# Autodesk Inventor assembly: X-axis assy
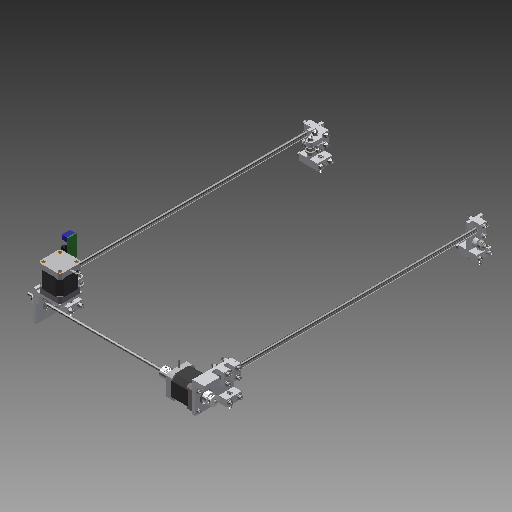
[picture p0: Inventor's stored thumbnail of the model, 512x512]
Saved by Autodesk Inventor 2018 (Build 220112000, 112)
## iProperties
Created: 2017-10-27
Part Number: X-axis assy
Document SubType Name: Assembly
Designer: Gabriel Smolnycki
Author: Gabriel Smolnycki
## Documents named in this file (13)
- E:\planb\mechanics\Subassemblies\X-axis assy.iam
- E:\planb\mechanics\Subassemblies\X-axis Idler 1 assy.iam
- E:\planb\mechanics\X-axis\X-axis Rod 8mm.ipt
- E:\planb\mechanics\Subassemblies\X-axis Motor Holder assy.iam
- E:\planb\mechanics\X-axis\X-axis Axle 5mm.ipt
- E:\planb\mechanics\Hardware\M4 SS Washer.ipt
- E:\planb\mechanics\Hardware\M4 SS Locknut.ipt
- E:\planb\mechanics\Hardware\M4x20 SS SHCS.ipt
- E:\planb\mechanics\Subassemblies\X-axis Y-axis Motor Holder assy.iam
- E:\planb\mechanics\Subassemblies\X-axis Driver Holder assy.iam
- E:\planb\mechanics\Hardware\T2.5 16T Pulley.ipt
- E:\planb\mechanics\Subassemblies\X-axis Idler 2 assy.iam
- E:\planb\mechanics\Hardware\5mm shaft coupler.ipt
## Components (18 placed, 12 different names)
1. X-axis Idler 1 assy:1 [sub-assembly] — Insert:1, Flush:1
2. X-axis Rod 8mm:1 — Insert:1, Insert:2
3. X-axis Motor Holder assy:1 [sub-assembly] — Insert:2, Flush:1, Insert:5, Flush:4, Insert:36
4. X-axis Axle 5mm:1 — Insert:5, Insert:38
5. X-axis Y-axis Motor Holder assy:1 [sub-assembly] — Insert:24, Insert:25, Insert:28, Insert:29
6. X-axis Driver Holder assy:1 [sub-assembly] — Insert:24, Insert:25, Flush:4, Insert:32, Insert:33, Insert:34, Insert:37
7. T2.5 16T Pulley:1 — Insert:37, Insert:38
8. M4 SS Washer:9 — Insert:28
9. M4x20 SS SHCS:2
10. M4 SS Washer:10 — Insert:29
11. M4x20 SS SHCS:1
12. M4 SS Washer:11 — Insert:32
13. M4 SS Locknut:5
14. M4 SS Washer:12 — Insert:33
15. M4 SS Locknut:6
16. X-axis Rod 8mm:2 — Insert:34, Insert:35
17. X-axis Idler 2 assy:1 [sub-assembly] — Insert:35
18. 5mm shaft coupler:1 — Insert:36
## Relationships (20: Insert 18, Flush 2)
- Insert:1 (-8 mm): X-axis Idler 1 assy:1 ↔ X-axis Rod 8mm:1
- Insert:2: X-axis Rod 8mm:1 ↔ X-axis Motor Holder assy:1
- Flush:1: X-axis Idler 1 assy:1 ↔ X-axis Motor Holder assy:1
- Insert:5: X-axis Motor Holder assy:1 ↔ X-axis Axle 5mm:1
- Insert:24: X-axis Y-axis Motor Holder assy:1 ↔ X-axis Driver Holder assy:1
- Insert:25: X-axis Y-axis Motor Holder assy:1 ↔ X-axis Driver Holder assy:1
- Flush:4: X-axis Motor Holder assy:1 ↔ X-axis Driver Holder assy:1
- [Insert]: M4 SS Washer:9 ↔ M4x20 SS SHCS:2
- [Insert]: M4 SS Washer:10 ↔ M4x20 SS SHCS:1
- Insert:28: X-axis Y-axis Motor Holder assy:1 ↔ M4 SS Washer:9
- Insert:29: X-axis Y-axis Motor Holder assy:1 ↔ M4 SS Washer:10
- [Insert]: M4 SS Washer:11 ↔ M4 SS Locknut:5
- [Insert]: M4 SS Washer:12 ↔ M4 SS Locknut:6
- Insert:32: X-axis Driver Holder assy:1 ↔ M4 SS Washer:11
- Insert:33: X-axis Driver Holder assy:1 ↔ M4 SS Washer:12
- Insert:34: X-axis Driver Holder assy:1 ↔ X-axis Rod 8mm:2
- Insert:35 (8 mm): X-axis Rod 8mm:2 ↔ X-axis Idler 2 assy:1
- Insert:36 (-12.4 mm): X-axis Motor Holder assy:1 ↔ 5mm shaft coupler:1
- Insert:37: X-axis Driver Holder assy:1 ↔ T2.5 16T Pulley:1
- Insert:38 (13.5 mm): X-axis Axle 5mm:1 ↔ T2.5 16T Pulley:1
## Named parameters: d38_d23_d17 = 0 mm, d39_d38_d23_d17 = 0 mm, d42_d24_d18 = 0 mm, d43_d24_d18 = 0 mm
